# Autodesk Inventor assembly: Assembly4
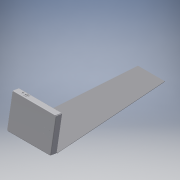
[picture p0: Inventor's stored thumbnail of the model, 180x180]
Saved by Autodesk Inventor 2016 (Build 200138000, 138)
## iProperties
Created: 2017-03-16
Part Number: Assembly4
Document SubType Name: Assembly
Designer: earlyp
Author: earlyp
## Documents named in this file (3)
- \\mps\fs\StudentHome\Student2018\earlyp\My Documents\Assembly4.iam
- H:\My Documents\peter early robot base.ipt
- H:\My Documents\robot side.ipt
## Components (2 placed, 2 different names)
1. peter early robot base:1 — Rigid:1
2. robot side:1 — Rigid:1
## Relationships (1: WeldJoint 1)
- Rigid:1 [WeldJoint]: peter early robot base:1 ↔ robot side:1
